# Autodesk Inventor assembly: Robot Frame '16
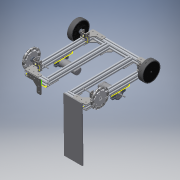
[picture p0: Inventor's stored thumbnail of the model, 180x180]
Saved by Autodesk Inventor 2017 (Build 210142000, 142)
## iProperties
Created: 2016-10-08
Part Number: Robot Frame '16
Document SubType Name: Assembly
Designer: Aditya
Author: Aditya
## Documents named in this file (17)
- C:\Users\Aditya\Documents\GitHub\RobotuxCAD\Team Robotux 15-16 Robot Cad Assets\Robot Frame '16.iam
- C:\Users\Aditya\Documents\GitHub\RobotuxCAD\Team Robotux 15-16 Robot Cad Assets\Andy Mark Parts\11.5in 1in alu ext.ipt
- C:\Users\Aditya\Documents\GitHub\RobotuxCAD\Team Robotux 15-16 Robot Cad Assets\Andy Mark Parts\15in 1in alu ext.ipt
- C:\Users\Aditya\Documents\GitHub\RobotuxCAD\Team Robotux 15-16 Robot Cad Assets\Andy Mark Parts\13in 1in alu ext.ipt
- C:\Users\Aditya\Documents\GitHub\RobotuxCAD\Team Robotux 15-16 Robot Cad Assets\Andy Mark Parts\3.7 in 1 in ext.ipt
- C:\Users\Aditya\Documents\GitHub\RobotuxCAD\Team Robotux 15-16 Robot Cad Assets\Andy Mark Parts\1in corner bracket for extrusions.ipt
- C:\Users\Aditya\Documents\GitHub\RobotuxCAD\Team Robotux 15-16 Robot Cad Assets\Andy Mark Parts\1in corner bracket for extrusions cut.ipt
- C:\Users\Aditya\Documents\GitHub\RobotuxCAD\Team Robotux 15-16 Robot Cad Assets\Andy Mark Parts\Inline Cylinder Mount Bracket.ipt
- C:\Users\Aditya\Documents\GitHub\RobotuxCAD\Team Robotux 15-16 Robot Cad Assets\Tetrix Parts\tetrix_739091_2013.ipt
- C:\Users\Aditya\Documents\GitHub\RobotuxCAD\Team Robotux 15-16 Robot Cad Assets\Tetrix Parts\tetrix_739088_2013.ipt
- C:\Users\Aditya\Documents\GitHub\RobotuxCAD\Team Robotux 15-16 Robot Cad Assets\Drive Motor Plate.ipt
- C:\Users\Aditya\Documents\GitHub\RobotuxCAD\Team Robotux 15-16 Robot Cad Assets\Tetrix Parts\tetrix_739089_2012.ipt
- C:\Users\Aditya\Documents\GitHub\RobotuxCAD\Team Robotux 15-16 Robot Cad Assets\Andy Mark Parts\am-2964NeveRest.ipt
- C:\Users\Aditya\Documents\GitHub\RobotuxCAD\Team Robotux 15-16 Robot Cad Assets\Tetrix Parts\tetrix_739172_2012.ipt
- C:\Users\Aditya\Documents\GitHub\RobotuxCAD\Team Robotux 15-16 Robot Cad Assets\Tetrix Parts\tetrix_736466_2012.ipt
- C:\Users\Aditya\Documents\GitHub\RobotuxCAD\Team Robotux 15-16 Robot Cad Assets\Andy Mark Parts\am-2648_4inWheel8mmHub.ipt
- C:\Users\Aditya\Documents\GitHub\RobotuxCAD\Team Robotux 15-16 Robot Cad Assets\pl8.ipt
## Components (51 placed, 16 different names)
1. 11.5in 1in alu ext:1 — Mate:1, Flush:1, Flush:2, Mate:2, Flush:3, Flush:4, Flush:33, Mate:18, Flush:35, Flush:38, Flush:40, Flush:50, Mate:26, Flush:51
2. 15in 1in alu ext:1 — Mate:2, Flush:3, Flush:4, Mate:4, Flush:7, Flush:8, Mate:23, Flush:46, Mate:24, Flush:47, Mate:25, Flush:49, Flush:52, Mate:30, Mate:32, Mate:36, Mate:38, Mate:59, Mate:60, Flush:53, Flush:54
3. 15in 1in alu ext:2 — Mate:1, Flush:1, Flush:2, Mate:3, Flush:5, Flush:6, Mate:19, Flush:37, Mate:20, Flush:39, Mate:21, Flush:41, Flush:44, Mate:27, Mate:29, Mate:33, Mate:35, Mate:61, Mate:62, Flush:55, Flush:56
4. 13in 1in alu ext:1 — Mate:5, Flush:9, Flush:10, Flush:32, Mate:17, Flush:34
5. 13in 1in alu ext:2 — Mate:6, Flush:11, Flush:12, Mate:15, Flush:30, Flush:36
6. 3.7 in 1 in ext:1 — Mate:4, Flush:7, Flush:8, Mate:5, Flush:9, Flush:10, Mate:16, Flush:31, Flush:45, Flush:48, Mate:87
7. 3.7 in 1 in ext:2 — Mate:3, Flush:5, Flush:6, Mate:6, Flush:11, Flush:12, Flush:29, Flush:42, Mate:22, Flush:43, Mate:88, Flush:64, Mate:89
8. 1in corner bracket for extrusions:1 — Mate:20, Flush:39, Flush:40, Mate:34
9. 1in corner bracket for extrusions:2 — Mate:24, Flush:47, Flush:48, Mate:31, Flush:63
10. 1in corner bracket for extrusions:3 — Mate:22, Flush:43, Flush:44, Mate:28
11. 1in corner bracket for extrusions:4 — Mate:26, Flush:51, Flush:52, Mate:37
12. 1in corner bracket for extrusions:5 — Mate:25, Flush:49, Flush:50
13. 1in corner bracket for extrusions:6 — Mate:19, Flush:37, Flush:38
14. 1in corner bracket for extrusions:7 — Mate:21, Flush:41, Flush:42
15. 1in corner bracket for extrusions:8 — Mate:23, Flush:45, Flush:46
16. 1in corner bracket for extrusions cut:1 — Mate:17, Flush:33, Flush:34
17. 1in corner bracket for extrusions cut:2 — Mate:15, Flush:29, Flush:30
18. 1in corner bracket for extrusions cut:3 — Mate:18, Flush:35, Flush:36
19. 1in corner bracket for extrusions cut:4 — Mate:16, Flush:31, Flush:32
20. Inline Cylinder Mount Bracket:1 — Mate:27, Mate:28, Mate:29, Mate:47, Mate:48, Mate:49, Mate:50
21. Inline Cylinder Mount Bracket:2 — Mate:33, Mate:34, Mate:35, Mate:51, Mate:52, Mate:53, Mate:54, Mate:57
22. Inline Cylinder Mount Bracket:3 — Mate:30, Mate:31, Mate:32, Mate:39, Mate:40, Mate:41, Mate:42
23. Inline Cylinder Mount Bracket:4 — Mate:36, Mate:37, Mate:38, Mate:43, Mate:44, Mate:45, Mate:46, Mate:58
24. tetrix_739091_2013:1 — Mate:51, Mate:52
25. tetrix_739091_2013:2 — Mate:43, Mate:44
26. tetrix_739091_2013:3 — Mate:39, Mate:40, Mate:55
27. tetrix_739091_2013:4 — Mate:49, Mate:50, Mate:56
28. tetrix_739091_2013:5 — Mate:47, Mate:48
29. tetrix_739091_2013:6 — Mate:45, Mate:46
30. tetrix_739091_2013:7 — Mate:53, Mate:54
31. tetrix_739091_2013:8 — Mate:41, Mate:42
32. tetrix_739088_2013:1 — Mate:55, Mate:83, Flush:59
33. tetrix_739088_2013:2 — Mate:56, Mate:84, Flush:60
34. tetrix_739088_2013:3 — Mate:57, Mate:85, Flush:61
35. tetrix_739088_2013:4 — Mate:58, Mate:86, Flush:62
36. Drive Motor Plate:1 — Mate:61, Mate:62, Flush:55, Flush:56, Mate:63, Mate:65, Mate:66
37. Drive Motor Plate:2 — Mate:59, Mate:60, Flush:53, Flush:54, Mate:64, Mate:67, Mate:68
38. tetrix_739089_2012:1 — Mate:64, Mate:67, Mate:68, Flush:58, Mate:70
39. tetrix_739089_2012:2 — Mate:63, Mate:65, Mate:66, Mate:69, Flush:57
40. am-2964NeveRest:1 — Flush:58, Mate:70
41. am-2964NeveRest:2 — Mate:69, Flush:57
42. tetrix_739172_2012:1 — Mate:74, Mate:75, Mate:76, Mate:84
43. tetrix_739172_2012:2 — Mate:80, Mate:81, Mate:82, Mate:85
44. tetrix_739172_2012:3 — Mate:71, Mate:72, Mate:73, Mate:83
45. tetrix_739172_2012:4 — Mate:77, Mate:78, Mate:79, Mate:86
46. tetrix_736466_2012:1 — Mate:71, Mate:72, Mate:73, Flush:59
47. tetrix_736466_2012:2 — Mate:74, Mate:75, Mate:76, Flush:60
48. am-2648_4inWheel8mmHub:1 — Mate:77, Mate:78, Mate:79, Flush:62
49. am-2648_4inWheel8mmHub:2 — Mate:80, Mate:81, Mate:82, Flush:61
50. pl8:1 — Mate:87, Flush:63
51. 1in corner bracket for extrusions:9 — Mate:88, Flush:64, Mate:89
## Relationships (129: Mate 81, Flush 48)
- Mate:1: 11.5in 1in alu ext:1 ↔ 15in 1in alu ext:2
- Flush:1: 11.5in 1in alu ext:1 ↔ 15in 1in alu ext:2
- Flush:2: 11.5in 1in alu ext:1 ↔ 15in 1in alu ext:2
- Mate:2: 11.5in 1in alu ext:1 ↔ 15in 1in alu ext:1
- Flush:3: 11.5in 1in alu ext:1 ↔ 15in 1in alu ext:1
- Flush:4: 11.5in 1in alu ext:1 ↔ 15in 1in alu ext:1
- Mate:3: 15in 1in alu ext:2 ↔ 3.7 in 1 in ext:2
- Flush:5: 15in 1in alu ext:2 ↔ 3.7 in 1 in ext:2
- Flush:6: 15in 1in alu ext:2 ↔ 3.7 in 1 in ext:2
- Mate:4: 15in 1in alu ext:1 ↔ 3.7 in 1 in ext:1
- Flush:7: 15in 1in alu ext:1 ↔ 3.7 in 1 in ext:1
- Flush:8: 15in 1in alu ext:1 ↔ 3.7 in 1 in ext:1
- Mate:5: 13in 1in alu ext:1 ↔ 3.7 in 1 in ext:1
- Flush:9: 13in 1in alu ext:1 ↔ 3.7 in 1 in ext:1
- Flush:10: 13in 1in alu ext:1 ↔ 3.7 in 1 in ext:1
- Mate:6: 13in 1in alu ext:2 ↔ 3.7 in 1 in ext:2
- Flush:11: 13in 1in alu ext:2 ↔ 3.7 in 1 in ext:2
- Flush:12: 13in 1in alu ext:2 ↔ 3.7 in 1 in ext:2
- Mate:15: 13in 1in alu ext:2 ↔ 1in corner bracket for extrusions cut:2
- Flush:29: 3.7 in 1 in ext:2 ↔ 1in corner bracket for extrusions cut:2
- Flush:30: 13in 1in alu ext:2 ↔ 1in corner bracket for extrusions cut:2
- Mate:16: 3.7 in 1 in ext:1 ↔ 1in corner bracket for extrusions cut:4
- Flush:31: 3.7 in 1 in ext:1 ↔ 1in corner bracket for extrusions cut:4
- Flush:32: 13in 1in alu ext:1 ↔ 1in corner bracket for extrusions cut:4
- Mate:17: 13in 1in alu ext:1 ↔ 1in corner bracket for extrusions cut:1
- Flush:33: 11.5in 1in alu ext:1 ↔ 1in corner bracket for extrusions cut:1
- Flush:34: 13in 1in alu ext:1 ↔ 1in corner bracket for extrusions cut:1
- Mate:18: 11.5in 1in alu ext:1 ↔ 1in corner bracket for extrusions cut:3
- Flush:35: 11.5in 1in alu ext:1 ↔ 1in corner bracket for extrusions cut:3
- Flush:36: 13in 1in alu ext:2 ↔ 1in corner bracket for extrusions cut:3
- Mate:19: 15in 1in alu ext:2 ↔ 1in corner bracket for extrusions:6
- Flush:37: 15in 1in alu ext:2 ↔ 1in corner bracket for extrusions:6
- Flush:38: 11.5in 1in alu ext:1 ↔ 1in corner bracket for extrusions:6
- Mate:20: 15in 1in alu ext:2 ↔ 1in corner bracket for extrusions:1
- Flush:39: 15in 1in alu ext:2 ↔ 1in corner bracket for extrusions:1
- Flush:40: 11.5in 1in alu ext:1 ↔ 1in corner bracket for extrusions:1
- Mate:21: 15in 1in alu ext:2 ↔ 1in corner bracket for extrusions:7
- Flush:41: 15in 1in alu ext:2 ↔ 1in corner bracket for extrusions:7
- Flush:42: 3.7 in 1 in ext:2 ↔ 1in corner bracket for extrusions:7
- Mate:22: 3.7 in 1 in ext:2 ↔ 1in corner bracket for extrusions:3
- Flush:43: 3.7 in 1 in ext:2 ↔ 1in corner bracket for extrusions:3
- Flush:44: 15in 1in alu ext:2 ↔ 1in corner bracket for extrusions:3
- Mate:23: 15in 1in alu ext:1 ↔ 1in corner bracket for extrusions:8
- Flush:45: 3.7 in 1 in ext:1 ↔ 1in corner bracket for extrusions:8
- Flush:46: 15in 1in alu ext:1 ↔ 1in corner bracket for extrusions:8
- Mate:24: 15in 1in alu ext:1 ↔ 1in corner bracket for extrusions:2
- Flush:47: 15in 1in alu ext:1 ↔ 1in corner bracket for extrusions:2
- Flush:48: 3.7 in 1 in ext:1 ↔ 1in corner bracket for extrusions:2
- Mate:25: 15in 1in alu ext:1 ↔ 1in corner bracket for extrusions:5
- Flush:49: 15in 1in alu ext:1 ↔ 1in corner bracket for extrusions:5
- Flush:50: 11.5in 1in alu ext:1 ↔ 1in corner bracket for extrusions:5
- Mate:26: 11.5in 1in alu ext:1 ↔ 1in corner bracket for extrusions:4
- Flush:51: 11.5in 1in alu ext:1 ↔ 1in corner bracket for extrusions:4
- Flush:52: 15in 1in alu ext:1 ↔ 1in corner bracket for extrusions:4
- Mate:27: 15in 1in alu ext:2 ↔ Inline Cylinder Mount Bracket:1
- Mate:28: 1in corner bracket for extrusions:3 ↔ Inline Cylinder Mount Bracket:1
- Mate:29: 15in 1in alu ext:2 ↔ Inline Cylinder Mount Bracket:1
- Mate:30: 15in 1in alu ext:1 ↔ Inline Cylinder Mount Bracket:3
- Mate:31: 1in corner bracket for extrusions:2 ↔ Inline Cylinder Mount Bracket:3
- Mate:32: 15in 1in alu ext:1 ↔ Inline Cylinder Mount Bracket:3
- Mate:33: 15in 1in alu ext:2 ↔ Inline Cylinder Mount Bracket:2
- Mate:34: 1in corner bracket for extrusions:1 ↔ Inline Cylinder Mount Bracket:2
- Mate:35: 15in 1in alu ext:2 ↔ Inline Cylinder Mount Bracket:2
- Mate:36: 15in 1in alu ext:1 ↔ Inline Cylinder Mount Bracket:4
- Mate:37: 1in corner bracket for extrusions:4 ↔ Inline Cylinder Mount Bracket:4
- Mate:38: 15in 1in alu ext:1 ↔ Inline Cylinder Mount Bracket:4
- Mate:39: Inline Cylinder Mount Bracket:3 ↔ tetrix_739091_2013:3
- Mate:40: Inline Cylinder Mount Bracket:3 ↔ tetrix_739091_2013:3
- Mate:41: Inline Cylinder Mount Bracket:3 ↔ tetrix_739091_2013:8
- Mate:42: Inline Cylinder Mount Bracket:3 ↔ tetrix_739091_2013:8
- Mate:43: Inline Cylinder Mount Bracket:4 ↔ tetrix_739091_2013:2
- Mate:44: Inline Cylinder Mount Bracket:4 ↔ tetrix_739091_2013:2
- Mate:45: Inline Cylinder Mount Bracket:4 ↔ tetrix_739091_2013:6
- Mate:46: Inline Cylinder Mount Bracket:4 ↔ tetrix_739091_2013:6
- Mate:47: Inline Cylinder Mount Bracket:1 ↔ tetrix_739091_2013:5
- Mate:48: Inline Cylinder Mount Bracket:1 ↔ tetrix_739091_2013:5
- Mate:49: Inline Cylinder Mount Bracket:1 ↔ tetrix_739091_2013:4
- Mate:50: Inline Cylinder Mount Bracket:1 ↔ tetrix_739091_2013:4
- Mate:51: Inline Cylinder Mount Bracket:2 ↔ tetrix_739091_2013:1
- Mate:52: Inline Cylinder Mount Bracket:2 ↔ tetrix_739091_2013:1
- Mate:53: Inline Cylinder Mount Bracket:2 ↔ tetrix_739091_2013:7
- Mate:54: Inline Cylinder Mount Bracket:2 ↔ tetrix_739091_2013:7
- Mate:55: tetrix_739091_2013:3 ↔ tetrix_739088_2013:1
- Mate:56: tetrix_739091_2013:4 ↔ tetrix_739088_2013:2
- Mate:57: Inline Cylinder Mount Bracket:2 ↔ tetrix_739088_2013:3
- Mate:58: Inline Cylinder Mount Bracket:4 ↔ tetrix_739088_2013:4
- Mate:59: 15in 1in alu ext:1 ↔ Drive Motor Plate:2
- Mate:60: 15in 1in alu ext:1 ↔ Drive Motor Plate:2
- Flush:53: 15in 1in alu ext:1 ↔ Drive Motor Plate:2
- Flush:54: 15in 1in alu ext:1 ↔ Drive Motor Plate:2
- Mate:61: 15in 1in alu ext:2 ↔ Drive Motor Plate:1
- Mate:62: 15in 1in alu ext:2 ↔ Drive Motor Plate:1
- Flush:55: 15in 1in alu ext:2 ↔ Drive Motor Plate:1
- Flush:56: 15in 1in alu ext:2 ↔ Drive Motor Plate:1
- Mate:63: Drive Motor Plate:1 ↔ tetrix_739089_2012:2
- Mate:64: Drive Motor Plate:2 ↔ tetrix_739089_2012:1
- Mate:65: Drive Motor Plate:1 ↔ tetrix_739089_2012:2
- Mate:66: Drive Motor Plate:1 ↔ tetrix_739089_2012:2
- Mate:67: Drive Motor Plate:2 ↔ tetrix_739089_2012:1
- Mate:68: Drive Motor Plate:2 ↔ tetrix_739089_2012:1
- Mate:69: tetrix_739089_2012:2 ↔ am-2964NeveRest:2
- Flush:57: tetrix_739089_2012:2 ↔ am-2964NeveRest:2
- Flush:58: tetrix_739089_2012:1 ↔ am-2964NeveRest:1
- Mate:70: tetrix_739089_2012:1 ↔ am-2964NeveRest:1
- Mate:71: tetrix_739172_2012:3 ↔ tetrix_736466_2012:1
- Mate:72: tetrix_739172_2012:3 ↔ tetrix_736466_2012:1
- Mate:73: tetrix_739172_2012:3 ↔ tetrix_736466_2012:1
- Mate:74: tetrix_739172_2012:1 ↔ tetrix_736466_2012:2
- Mate:75: tetrix_739172_2012:1 ↔ tetrix_736466_2012:2
- Mate:76: tetrix_739172_2012:1 ↔ tetrix_736466_2012:2
- Mate:77: tetrix_739172_2012:4 ↔ am-2648_4inWheel8mmHub:1
- Mate:78: tetrix_739172_2012:4 ↔ am-2648_4inWheel8mmHub:1
- Mate:79: tetrix_739172_2012:4 ↔ am-2648_4inWheel8mmHub:1
- Mate:80: tetrix_739172_2012:2 ↔ am-2648_4inWheel8mmHub:2
- Mate:81: tetrix_739172_2012:2 ↔ am-2648_4inWheel8mmHub:2
- Mate:82: tetrix_739172_2012:2 ↔ am-2648_4inWheel8mmHub:2
- Mate:83: tetrix_739088_2013:1 ↔ tetrix_739172_2012:3
- Flush:59: tetrix_739088_2013:1 ↔ tetrix_736466_2012:1
- Mate:84: tetrix_739088_2013:2 ↔ tetrix_739172_2012:1
- Flush:60: tetrix_739088_2013:2 ↔ tetrix_736466_2012:2
- Mate:85: tetrix_739088_2013:3 ↔ tetrix_739172_2012:2
- Flush:61: tetrix_739088_2013:3 ↔ am-2648_4inWheel8mmHub:2
- Mate:86: tetrix_739088_2013:4 ↔ tetrix_739172_2012:4
- Flush:62: tetrix_739088_2013:4 ↔ am-2648_4inWheel8mmHub:1
- Mate:87: 3.7 in 1 in ext:1 ↔ pl8:1
- Flush:63: 1in corner bracket for extrusions:2 ↔ pl8:1
- Mate:88: 3.7 in 1 in ext:2 ↔ 1in corner bracket for extrusions:9
- Flush:64: 3.7 in 1 in ext:2 ↔ 1in corner bracket for extrusions:9
- Mate:89: 3.7 in 1 in ext:2 ↔ 1in corner bracket for extrusions:9
